# Autodesk Inventor assembly: Bikair
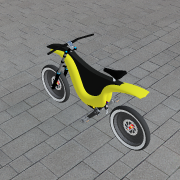
[picture p0: Inventor's stored thumbnail of the model, 180x180]
Saved by Autodesk Inventor 2016 (Build 200138000, 138)
## iProperties
Created: 2015-03-25
Part Number: Bikair
Document SubType Name: Assembly
Designer: Yann
Author: Yann
## Documents named in this file (10)
- C:\Users\Yann\Documents\GitHub\BIKAIR_CAD\Source\Bikair.iam
- C:\Users\Yann\Documents\GitHub\BIKAIR_CAD\Source\Frame\Frame.iam
- C:\Users\Yann\Documents\GitHub\BIKAIR_CAD\Source\Energy_Pack\Energy_Pack.iam
- C:\Users\Yann\Documents\GitHub\BIKAIR_CAD\Source\Motor\Motor.iam
- C:\Users\Yann\Documents\GitHub\BIKAIR_CAD\Source\Rear_Train\Rear_Train.iam
- C:\Users\Yann\Documents\GitHub\BIKAIR_CAD\Source\Rear_Train\Wheel\wheel.iam
- C:\Users\Yann\Documents\GitHub\BIKAIR_CAD\Source\Front_Train\Front_Train.iam
- C:\Users\Yann\Documents\GitHub\BIKAIR_CAD\Source\Bike_Drive\Bike_Drive.iam
- C:\Users\Yann\Documents\GitHub\BIKAIR_CAD\Source\User\ERGOMAN POST.iam
- C:\Users\Yann\Documents\GitHub\BIKAIR_CAD\Source\Motor\Colossus_7kW.iam
## Components (12 placed, 9 different names)
1. Frame:1 [sub-assembly] — Affleurement:1, Placage:1, Placage:2
2. Energy_Pack:1 [sub-assembly] — Affleurement:2, Angle:1
3. Motor:1 [sub-assembly] — Placage:3
4. Rear_Train:1 [sub-assembly] — Affleurement:7
5. wheel:1 [sub-assembly] — Affleurement:5
6. wheel:3 [sub-assembly]
7. Front_Train:1 [sub-assembly] — Placage:5, Affleurement:8, Angle:4
8. Motor:2 [sub-assembly] — Placage:6
9. Bike_Drive:1 [sub-assembly] — Placage:10
10. ERGOMAN POST:1 [sub-assembly] — Affleurement:9
11. Colossus_7kW:1 [sub-assembly]
12. Colossus_7kW:2 [sub-assembly]
## Relationships (18: Flush 7, Mate 7, Angle 4)
- Affleurement:1 [Flush]: Frame:1
- Placage:1 [Mate]: Frame:1
- Placage:2 [Mate]: Frame:1
- Affleurement:2 [Flush]: Energy_Pack:1
- Angle:1 (5 deg): Energy_Pack:1
- Placage:3 [Mate] (40 mm): Motor:1
- Affleurement:5 [Flush]: wheel:1
- [Mate]: Front_Train:1
- [Angle] (22 deg): Front_Train:1
- [Flush]: Front_Train:1
- [Angle] (155 deg): Front_Train:1
- Affleurement:7 [Flush]: Rear_Train:1
- Placage:5 [Mate]: Front_Train:1
- Affleurement:8 [Flush]: Front_Train:1
- Angle:4 (25 deg): Front_Train:1
- Placage:6 [Mate]: Motor:2
- Placage:10 [Mate] (-50 mm): Bike_Drive:1
- Affleurement:9 [Flush]: ERGOMAN POST:1
